# Autodesk Inventor assembly: Tip
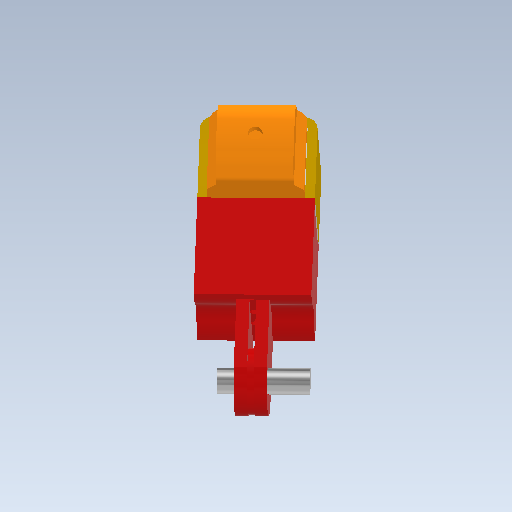
[picture p0: Inventor's stored thumbnail of the model, 512x512]
Saved by Autodesk Inventor 2020 (Build 240168000, 168)
## iProperties
Created: 2020-02-17
Part Number: Tip
Document SubType Name: Assembly
Designer: PROXS
Author: PROXS
## Documents named in this file (7)
- C:\Users\sami_\Documents\V1.6\Workgroups\NotInProject\THUMB\Assembly\Tip.iam
- C:\Users\sami_\Documents\V1.6\Workgroups\NotInProject\THUMB\Assembly\fingertip lid 4.ipt
- C:\Users\sami_\Documents\V1.6\Workgroups\NotInProject\INDEX\fingertip skeleton 5.ipt
- C:\Users\sami_\Documents\V1.6\Workgroups\NotInProject\INDEX\fingertip lid 5.ipt
- C:\Users\sami_\Documents\V1.6\Workgroups\NotInProject\SHAFT.ipt
- C:\Users\sami_\Documents\V1.6\Workgroups\NotInProject\THUMB\L3.ipt
- C:\Users\sami_\Documents\V1.6\Workgroups\NotInProject\Fingertiptest2-Solid 2mm base.ipt
## Components (6 placed, 6 different names)
1. L3:1 — Rigid:3
2. fingertip skeleton 5:1 — Rigid:2, Rigid:3, Rigid:4
3. fingertip lid 5:1
4. fingertip lid 4:2 — Rigid:2
5. SHAFT:1
6. Fingertiptest2-Solid 2mm base:1 — Rigid:4
## Relationships (6: WeldJoint 4, Mate 2)
- [WeldJoint]: fingertip skeleton 5:1 ↔ fingertip lid 5:1
- Rigid:2 [WeldJoint]: fingertip skeleton 5:1 ↔ fingertip lid 4:2
- [Mate]: L3:1 ↔ SHAFT:1
- [Mate]: L3:1 ↔ SHAFT:1
- Rigid:3 [WeldJoint]: L3:1 ↔ fingertip skeleton 5:1
- Rigid:4 [WeldJoint] (-1 mm): fingertip skeleton 5:1 ↔ Fingertiptest2-Solid 2mm base:1
